# Autodesk Inventor assembly: Roof
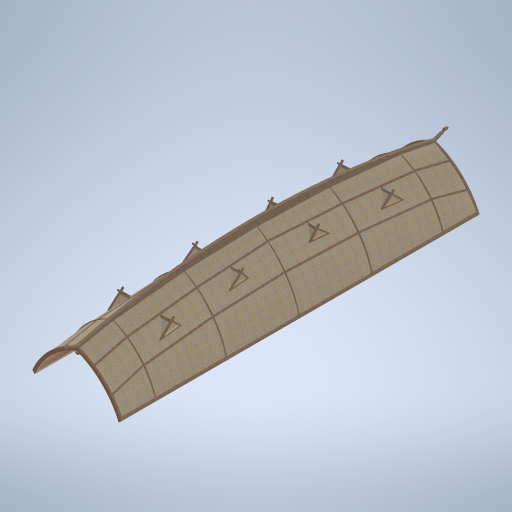
[picture p0: Inventor's stored thumbnail of the model, 512x512]
Saved by Autodesk Inventor 2024.2 (Build 282272000, 272)
## iProperties
Created: 2024-05-18
Part Number: Roof
Document SubType Name: Assembly
Designer: LOSTER_1
Author: LOSTER_1
## Documents named in this file (69)
- C:\Users\LOSTER_1\OneDrive\桌面\school\senior\Inventor_Project\ROOF\Roof.iam
- C:\Users\LOSTER_1\OneDrive\桌面\school\senior\Inventor_Project\ROOF\roof_beam.ipt
- C:\Users\LOSTER_1\OneDrive\桌面\school\senior\Inventor_Project\ROOF\gripping_beast.ipt
- C:\Users\LOSTER_1\OneDrive\桌面\school\senior\Inventor_Project\ROOF\main_crossbeam.ipt
- C:\Users\LOSTER_1\OneDrive\桌面\school\senior\Inventor_Project\ROOF\outer_curve_beam.ipt
- C:\Users\LOSTER_1\OneDrive\桌面\school\senior\Inventor_Project\ROOF\roof_straight_beam.ipt
- C:\Users\LOSTER_1\OneDrive\桌面\school\senior\Inventor_Project\ROOF\curve_beam_01.ipt
- C:\Users\LOSTER_1\OneDrive\桌面\school\senior\Inventor_Project\ROOF\curve_beam_02.ipt
- C:\Users\LOSTER_1\OneDrive\桌面\school\senior\Inventor_Project\ROOF\curve_beam_03.ipt
- C:\Users\LOSTER_1\OneDrive\桌面\school\senior\Inventor_Project\ROOF\support_beam_segments\support_beam_segment_0101.ipt
- C:\Users\LOSTER_1\OneDrive\桌面\school\senior\Inventor_Project\ROOF\support_beam_segments\support_beam_segment_0102.ipt
- C:\Users\LOSTER_1\OneDrive\桌面\school\senior\Inventor_Project\ROOF\support_beam_segments\support_beam_segment_0103.ipt
- C:\Users\LOSTER_1\OneDrive\桌面\school\senior\Inventor_Project\ROOF\support_beam_segments\support_beam_segment_0104.ipt
- C:\Users\LOSTER_1\OneDrive\桌面\school\senior\Inventor_Project\ROOF\support_beam_segments\support_beam_segment_0105.ipt
- C:\Users\LOSTER_1\OneDrive\桌面\school\senior\Inventor_Project\ROOF\support_beam_segments\support_beam_segment_0106.ipt
- C:\Users\LOSTER_1\OneDrive\桌面\school\senior\Inventor_Project\ROOF\support_beam_segments\support_beam_segment_0101_MIR.ipt
- C:\Users\LOSTER_1\OneDrive\桌面\school\senior\Inventor_Project\ROOF\support_beam_segments\support_beam_segment_0102_MIR.ipt
- C:\Users\LOSTER_1\OneDrive\桌面\school\senior\Inventor_Project\ROOF\support_beam_segments\support_beam_segment_0103_MIR.ipt
- C:\Users\LOSTER_1\OneDrive\桌面\school\senior\Inventor_Project\ROOF\support_beam_segments\support_beam_segment_0104_MIR.ipt
- C:\Users\LOSTER_1\OneDrive\桌面\school\senior\Inventor_Project\ROOF\support_beam_segments\support_beam_segment_0105_MIR.ipt
- C:\Users\LOSTER_1\OneDrive\桌面\school\senior\Inventor_Project\ROOF\support_beam_segments\support_beam_segment_0106_MIR.ipt
- C:\Users\LOSTER_1\OneDrive\桌面\school\senior\Inventor_Project\ROOF\support_beam_segments\support_beam_segment_0101_MIR1.ipt
- C:\Users\LOSTER_1\OneDrive\桌面\school\senior\Inventor_Project\ROOF\support_beam_segments\support_beam_segment_0102_MIR1.ipt
- C:\Users\LOSTER_1\OneDrive\桌面\school\senior\Inventor_Project\ROOF\support_beam_segments\support_beam_segment_0103_MIR1.ipt
- C:\Users\LOSTER_1\OneDrive\桌面\school\senior\Inventor_Project\ROOF\support_beam_segments\support_beam_segment_0104_MIR1.ipt
- C:\Users\LOSTER_1\OneDrive\桌面\school\senior\Inventor_Project\ROOF\support_beam_segments\support_beam_segment_0105_MIR1.ipt
- C:\Users\LOSTER_1\OneDrive\桌面\school\senior\Inventor_Project\ROOF\support_beam_segments\support_beam_segment_0106_MIR1.ipt
- C:\Users\LOSTER_1\OneDrive\桌面\school\senior\Inventor_Project\ROOF\support_beam_segments\support_beam_segment_0101_MIR_MIR.ipt
- C:\Users\LOSTER_1\OneDrive\桌面\school\senior\Inventor_Project\ROOF\support_beam_segments\support_beam_segment_0102_MIR_MIR.ipt
- C:\Users\LOSTER_1\OneDrive\桌面\school\senior\Inventor_Project\ROOF\support_beam_segments\support_beam_segment_0103_MIR_MIR.ipt
- C:\Users\LOSTER_1\OneDrive\桌面\school\senior\Inventor_Project\ROOF\support_beam_segments\support_beam_segment_0104_MIR_MIR.ipt
- C:\Users\LOSTER_1\OneDrive\桌面\school\senior\Inventor_Project\ROOF\support_beam_segments\support_beam_segment_0105_MIR_MIR.ipt
- C:\Users\LOSTER_1\OneDrive\桌面\school\senior\Inventor_Project\ROOF\support_beam_segments\support_beam_segment_0106_MIR_MIR.ipt
- C:\Users\LOSTER_1\OneDrive\桌面\school\senior\Inventor_Project\ROOF\panel_blocks\panel_block_03.ipt
- C:\Users\LOSTER_1\OneDrive\桌面\school\senior\Inventor_Project\ROOF\panel_blocks\panel_block_02.ipt
- C:\Users\LOSTER_1\OneDrive\桌面\school\senior\Inventor_Project\ROOF\panel_blocks\panel_block_01.ipt
- C:\Users\LOSTER_1\OneDrive\桌面\school\senior\Inventor_Project\ROOF\panel_blocks\panel_block_03_MIR.ipt
- C:\Users\LOSTER_1\OneDrive\桌面\school\senior\Inventor_Project\ROOF\panel_blocks\panel_block_02_MIR.ipt
- C:\Users\LOSTER_1\OneDrive\桌面\school\senior\Inventor_Project\ROOF\panel_blocks\panel_block_01_MIR.ipt
- C:\Users\LOSTER_1\OneDrive\桌面\school\senior\Inventor_Project\ROOF\panel_blocks\panel_block_03_MIR1.ipt
- C:\Users\LOSTER_1\OneDrive\桌面\school\senior\Inventor_Project\ROOF\panel_blocks\panel_block_01_MIR1.ipt
- C:\Users\LOSTER_1\OneDrive\桌面\school\senior\Inventor_Project\ROOF\panel_blocks\panel_block_03_MIR_MIR.ipt
- C:\Users\LOSTER_1\OneDrive\桌面\school\senior\Inventor_Project\ROOF\panel_blocks\panel_block_02_MIR_MIR.ipt
- C:\Users\LOSTER_1\OneDrive\桌面\school\senior\Inventor_Project\ROOF\panel_blocks\panel_block_01_MIR_MIR.ipt
- C:\Users\LOSTER_1\OneDrive\桌面\school\senior\Inventor_Project\ROOF\panel_blocks\panel_pad_02 .ipt
- C:\Users\LOSTER_1\OneDrive\桌面\school\senior\Inventor_Project\ROOF\panel_blocks\panel_block_02_MIR2.ipt
- C:\Users\LOSTER_1\OneDrive\桌面\school\senior\Inventor_Project\ROOF\panel_blocks\panel_pad_03.ipt
- C:\Users\LOSTER_1\OneDrive\桌面\school\senior\Inventor_Project\ROOF\panel_blocks\panel_pad_frame_01.ipt
- C:\Users\LOSTER_1\OneDrive\桌面\school\senior\Inventor_Project\ROOF\panel_blocks\panel_pad_frame_02.ipt
- C:\Users\LOSTER_1\OneDrive\桌面\school\senior\Inventor_Project\ROOF\panel_blocks\panel_pad_02 _MIR.ipt
- C:\Users\LOSTER_1\OneDrive\桌面\school\senior\Inventor_Project\ROOF\panel_blocks\panel_pad_03_MIR.ipt
- C:\Users\LOSTER_1\OneDrive\桌面\school\senior\Inventor_Project\ROOF\panel_blocks\panel_pad_frame_01_MIR.ipt
- C:\Users\LOSTER_1\OneDrive\桌面\school\senior\Inventor_Project\ROOF\panel_blocks\panel_pad_frame_02_MIR.ipt
- C:\Users\LOSTER_1\OneDrive\桌面\school\senior\Inventor_Project\ROOF\panel_blocks\panel_pad_02 _MIR1.ipt
- C:\Users\LOSTER_1\OneDrive\桌面\school\senior\Inventor_Project\ROOF\panel_blocks\panel_pad_03_MIR1.ipt
- C:\Users\LOSTER_1\OneDrive\桌面\school\senior\Inventor_Project\ROOF\panel_blocks\panel_pad_frame_01_MIR1.ipt
- C:\Users\LOSTER_1\OneDrive\桌面\school\senior\Inventor_Project\ROOF\panel_blocks\panel_pad_frame_02_MIR1.ipt
- C:\Users\LOSTER_1\OneDrive\桌面\school\senior\Inventor_Project\ROOF\panel_blocks\panel_pad_02 _MIR_MIR.ipt
- C:\Users\LOSTER_1\OneDrive\桌面\school\senior\Inventor_Project\ROOF\panel_blocks\panel_pad_03_MIR_MIR.ipt
- C:\Users\LOSTER_1\OneDrive\桌面\school\senior\Inventor_Project\ROOF\panel_blocks\panel_pad_frame_01_MIR_MIR.ipt
- C:\Users\LOSTER_1\OneDrive\桌面\school\senior\Inventor_Project\ROOF\panel_blocks\panel_pad_frame_02_MIR_MIR.ipt
- C:\Users\LOSTER_1\OneDrive\桌面\school\senior\Inventor_Project\ROOF\panel_blocks\pad_outframe_02.ipt
- C:\Users\LOSTER_1\OneDrive\桌面\school\senior\Inventor_Project\ROOF\panel_blocks\pad_outframe_03.ipt
- C:\Users\LOSTER_1\OneDrive\桌面\school\senior\Inventor_Project\ROOF\panel_blocks\pad_outframe_02_MIR.ipt
- C:\Users\LOSTER_1\OneDrive\桌面\school\senior\Inventor_Project\ROOF\panel_blocks\pad_outframe_03_MIR.ipt
- C:\Users\LOSTER_1\OneDrive\桌面\school\senior\Inventor_Project\ROOF\panel_blocks\pad_outframe_02_MIR1.ipt
- C:\Users\LOSTER_1\OneDrive\桌面\school\senior\Inventor_Project\ROOF\panel_blocks\pad_outframe_03_MIR1.ipt
- C:\Users\LOSTER_1\OneDrive\桌面\school\senior\Inventor_Project\ROOF\panel_blocks\pad_outframe_02_MIR_MIR.ipt
- C:\Users\LOSTER_1\OneDrive\桌面\school\senior\Inventor_Project\ROOF\panel_blocks\pad_outframe_03_MIR_MIR.ipt
## Components (80 placed, 68 different names)
1. roof_beam:1 — Mate:1, Mate:2, Mate:3, Mate:4, Mate:5, Mate:6, Mate:7, Mate:8, Mate:31, Mate:32, Mate:33, Mate:34, Mate:35, Mate:36, Mate:37, Mate:38, Mate:39, Mate:40, Mate:41, Mate:42, Mate:43, Mate:44, Mate:45, Mate:46, Mate:47, Mate:48, Mate:49, Mate:50, Mate:51, Mate:52, Mate:53, Mate:54, Mate:55, Flush:2
2. gripping_beast:1 — Mate:1, Mate:2, Mate:3, Mate:4
3. gripping_beast:2 — Mate:5
4. main_crossbeam:1 — Mate:6, Mate:7, Mate:8, Mate:11, Mate:14, Mate:19, Mate:20, Mate:21, Mate:22
5. outer_curve_beam:1 — Mate:9, Mate:10, Mate:11, Mate:12, Mate:13, Mate:26, Mate:28, Mate:56, Mate:57, Mate:58, Mate:59, Mate:60, Mate:74
6. outer_curve_beam:2 — Mate:9, Mate:10, Mate:12, Mate:13, Mate:14, Mate:29, Mate:30, Mate:75, Mate:76, Mate:77, Mate:78
7. outer_curve_beam:3 — Mate:23, Mate:24, Mate:25, Mate:27, Mate:79, Mate:80, Mate:81
8. outer_curve_beam:4 — Mate:19, Mate:20, Mate:21, Mate:22, Mate:23, Mate:24, Mate:25, Mate:82, Mate:83, Mate:84, Mate:85
9. roof_straight_beam:1 — Mate:26, Mate:27, Mate:28
10. roof_straight_beam:2 — Mate:29, Mate:30
11. curve_beam_01:1 — Mate:31, Mate:32, Mate:33
12. curve_beam_01:2 — Mate:34, Mate:35, Mate:61, Mate:63, Mate:64, Mate:65
13. curve_beam_01:3 — Mate:36, Mate:37
14. curve_beam_01:4 — Mate:38, Mate:39
15. curve_beam_02:1 — Mate:43, Mate:44
16. curve_beam_02:2 — Mate:40, Mate:41, Mate:42
17. curve_beam_02:3 — Mate:45, Mate:46, Mate:47, Mate:62, Mate:66, Mate:67, Mate:68, Mate:69, Mate:70
18. curve_beam_02:4 — Mate:48, Mate:49, Mate:50
19. curve_beam_03:1 — Mate:51, Mate:52, Flush:1
20. curve_beam_03:2 — Mate:53, Mate:54, Mate:55
21. support_beam_segment_0101:1 — Mate:56, Mate:57, Mate:58, Mate:73
22. support_beam_segment_0102:1 — Mate:59, Mate:60
23. support_beam_segment_0103:1 — Mate:61, Mate:62, Mate:71, Mate:72
24. support_beam_segment_0104:1 — Mate:63, Mate:64, Mate:65
25. support_beam_segment_0105:1 — Mate:66, Mate:67
26. support_beam_segment_0106:1 — Mate:68, Mate:69
27. support_beam_segment_0101_MIR:1 — Mate:80, Mate:81
28. support_beam_segment_0102_MIR:1 — Mate:79
29. support_beam_segment_0103_MIR:1
30. support_beam_segment_0104_MIR:1
31. support_beam_segment_0105_MIR:1
32. support_beam_segment_0106_MIR:1
33. support_beam_segment_0101_MIR1:1 — Mate:75, Mate:76
34. support_beam_segment_0102_MIR1:1 — Mate:77, Mate:78
35. support_beam_segment_0103_MIR1:1
36. support_beam_segment_0104_MIR1:1
37. support_beam_segment_0105_MIR1:1
38. support_beam_segment_0106_MIR1:1
39. support_beam_segment_0101_MIR_MIR:1 — Mate:82, Mate:83
40. support_beam_segment_0102_MIR_MIR:1 — Mate:84, Mate:85
41. support_beam_segment_0103_MIR_MIR:1
42. support_beam_segment_0104_MIR_MIR:1
43. support_beam_segment_0105_MIR_MIR:1
44. support_beam_segment_0106_MIR_MIR:1
45. panel_block_03:1 — Mate:70, Mate:87
46. panel_block_02:1 — Mate:71, Mate:72, Mate:86
47. panel_block_01:1 — Mate:73, Mate:74
48. panel_block_03_MIR:1
49. panel_block_02_MIR:1
50. panel_block_01_MIR:1
51. panel_block_03_MIR1:1
52. panel_block_01_MIR1:1
53. panel_block_03_MIR_MIR:1
54. panel_block_02_MIR_MIR:1
55. panel_block_01_MIR_MIR:1
56. panel_pad_02 :1 — Mate:86, Mate:88, Mate:96
57. panel_block_02_MIR2:1
58. panel_pad_03:1 — Mate:87, Mate:89
59. panel_pad_frame_01:1 — Mate:88
60. panel_pad_frame_02:1 — Mate:89, Mate:97
61. panel_pad_02 _MIR:1 — Mate:90
62. panel_pad_03_MIR:1 — Mate:91
63. panel_pad_frame_01_MIR:1 — Mate:90
64. panel_pad_frame_02_MIR:1 — Mate:91
65. panel_pad_02 _MIR1:1 — Mate:92
66. panel_pad_03_MIR1:1 — Mate:93
67. panel_pad_frame_01_MIR1:1 — Mate:92
68. panel_pad_frame_02_MIR1:1 — Mate:93
69. panel_pad_02 _MIR_MIR:1 — Mate:94
70. panel_pad_03_MIR_MIR:1 — Mate:95
71. panel_pad_frame_01_MIR_MIR:1 — Mate:94
72. panel_pad_frame_02_MIR_MIR:1 — Mate:95
73. pad_outframe_02:1 — Mate:96
74. pad_outframe_03:1 — Mate:97
75. pad_outframe_02_MIR:1
76. pad_outframe_03_MIR:1
77. pad_outframe_02_MIR1:1
78. pad_outframe_03_MIR1:1
79. pad_outframe_02_MIR_MIR:1
80. pad_outframe_03_MIR_MIR:1
## Relationships (99: Mate 97, Flush 2)
- Mate:1: roof_beam:1 ↔ gripping_beast:1
- Mate:2: roof_beam:1 ↔ gripping_beast:1
- Mate:3: roof_beam:1 ↔ gripping_beast:1
- Mate:4: roof_beam:1 ↔ gripping_beast:1
- Mate:5: roof_beam:1 ↔ gripping_beast:2
- Mate:6: roof_beam:1 ↔ main_crossbeam:1
- Mate:7: roof_beam:1 ↔ main_crossbeam:1
- Mate:8: roof_beam:1 ↔ main_crossbeam:1
- Mate:9: outer_curve_beam:1 ↔ outer_curve_beam:2
- Mate:10: outer_curve_beam:1 ↔ outer_curve_beam:2
- Mate:11: main_crossbeam:1 ↔ outer_curve_beam:1
- Mate:12: outer_curve_beam:1 ↔ outer_curve_beam:2
- Mate:13: outer_curve_beam:1 ↔ outer_curve_beam:2
- Mate:14: main_crossbeam:1 ↔ outer_curve_beam:2
- [Mate]: outer_curve_beam:3 ↔ outer_curve_beam:4
- [Mate]: outer_curve_beam:3 ↔ outer_curve_beam:4
- [Mate]: outer_curve_beam:3 ↔ outer_curve_beam:4
- [Mate]: outer_curve_beam:3 ↔ outer_curve_beam:4
- Mate:19: main_crossbeam:1 ↔ outer_curve_beam:4
- Mate:20: main_crossbeam:1 ↔ outer_curve_beam:4
- Mate:21: main_crossbeam:1 ↔ outer_curve_beam:4
- Mate:22: main_crossbeam:1 ↔ outer_curve_beam:4
- Mate:23: outer_curve_beam:3 ↔ outer_curve_beam:4
- Mate:24: outer_curve_beam:3 ↔ outer_curve_beam:4
- Mate:25: outer_curve_beam:3 ↔ outer_curve_beam:4
- Mate:26: outer_curve_beam:1 ↔ roof_straight_beam:1
- Mate:27: outer_curve_beam:3 ↔ roof_straight_beam:1
- Mate:28: outer_curve_beam:1 ↔ roof_straight_beam:1
- Mate:29: outer_curve_beam:2 ↔ roof_straight_beam:2
- Mate:30: outer_curve_beam:2 ↔ roof_straight_beam:2
- Mate:31: roof_beam:1 ↔ curve_beam_01:1
- Mate:32: roof_beam:1 ↔ curve_beam_01:1
- Mate:33: roof_beam:1 ↔ curve_beam_01:1
- Mate:34: roof_beam:1 ↔ curve_beam_01:2
- Mate:35: roof_beam:1 ↔ curve_beam_01:2
- Mate:36: roof_beam:1 ↔ curve_beam_01:3
- Mate:37: roof_beam:1 ↔ curve_beam_01:3
- Mate:38: roof_beam:1 ↔ curve_beam_01:4
- Mate:39: roof_beam:1 ↔ curve_beam_01:4
- Mate:40: roof_beam:1 ↔ curve_beam_02:2
- Mate:41: roof_beam:1 ↔ curve_beam_02:2
- Mate:42: roof_beam:1 ↔ curve_beam_02:2
- Mate:43: roof_beam:1 ↔ curve_beam_02:1
- Mate:44: roof_beam:1 ↔ curve_beam_02:1
- Mate:45: roof_beam:1 ↔ curve_beam_02:3
- Mate:46: roof_beam:1 ↔ curve_beam_02:3
- Mate:47: roof_beam:1 ↔ curve_beam_02:3
- Mate:48: roof_beam:1 ↔ curve_beam_02:4
- Mate:49: roof_beam:1 ↔ curve_beam_02:4
- Mate:50: roof_beam:1 ↔ curve_beam_02:4
- Mate:51: roof_beam:1 ↔ curve_beam_03:1
- Mate:52: roof_beam:1 ↔ curve_beam_03:1
- Mate:53: roof_beam:1 ↔ curve_beam_03:2
- Mate:54: roof_beam:1 ↔ curve_beam_03:2
- Mate:55: roof_beam:1 ↔ curve_beam_03:2
- Mate:56: outer_curve_beam:1 ↔ support_beam_segment_0101:1
- Mate:57: outer_curve_beam:1 ↔ support_beam_segment_0101:1
- Mate:58: outer_curve_beam:1 ↔ support_beam_segment_0101:1
- Mate:59: outer_curve_beam:1 ↔ support_beam_segment_0102:1
- Mate:60: outer_curve_beam:1 ↔ support_beam_segment_0102:1
- Mate:61: curve_beam_01:2 ↔ support_beam_segment_0103:1
- Mate:62: curve_beam_02:3 ↔ support_beam_segment_0103:1
- Mate:63: curve_beam_01:2 ↔ support_beam_segment_0104:1
- Mate:64: curve_beam_01:2 ↔ support_beam_segment_0104:1
- Mate:65: curve_beam_01:2 ↔ support_beam_segment_0104:1
- Mate:66: curve_beam_02:3 ↔ support_beam_segment_0105:1
- Mate:67: curve_beam_02:3 ↔ support_beam_segment_0105:1
- Mate:68: curve_beam_02:3 ↔ support_beam_segment_0106:1
- Mate:69: curve_beam_02:3 ↔ support_beam_segment_0106:1
- Flush:1 (-50 mm): curve_beam_03:1
- Flush:2 (-150 mm): roof_beam:1
- Mate:70: curve_beam_02:3 ↔ panel_block_03:1
- Mate:71: support_beam_segment_0103:1 ↔ panel_block_02:1
- Mate:72: support_beam_segment_0103:1 ↔ panel_block_02:1
- Mate:73: support_beam_segment_0101:1 ↔ panel_block_01:1
- Mate:74: outer_curve_beam:1 ↔ panel_block_01:1
- Mate:75: outer_curve_beam:2 ↔ support_beam_segment_0101_MIR1:1
- Mate:76: outer_curve_beam:2 ↔ support_beam_segment_0101_MIR1:1
- Mate:77: outer_curve_beam:2 ↔ support_beam_segment_0102_MIR1:1
- Mate:78: outer_curve_beam:2 ↔ support_beam_segment_0102_MIR1:1
- Mate:79: outer_curve_beam:3 ↔ support_beam_segment_0102_MIR:1
- Mate:80: outer_curve_beam:3 ↔ support_beam_segment_0101_MIR:1
- Mate:81: outer_curve_beam:3 ↔ support_beam_segment_0101_MIR:1
- Mate:82: outer_curve_beam:4 ↔ support_beam_segment_0101_MIR_MIR:1
- Mate:83: outer_curve_beam:4 ↔ support_beam_segment_0101_MIR_MIR:1
- Mate:84: outer_curve_beam:4 ↔ support_beam_segment_0102_MIR_MIR:1
- Mate:85: outer_curve_beam:4 ↔ support_beam_segment_0102_MIR_MIR:1
- Mate:86: panel_block_02:1 ↔ panel_pad_02 :1
- Mate:87: panel_block_03:1 ↔ panel_pad_03:1
- Mate:88: panel_pad_02 :1 ↔ panel_pad_frame_01:1
- Mate:89: panel_pad_03:1 ↔ panel_pad_frame_02:1
- Mate:90: panel_pad_02 _MIR:1 ↔ panel_pad_frame_01_MIR:1
- Mate:91: panel_pad_03_MIR:1 ↔ panel_pad_frame_02_MIR:1
- Mate:92: panel_pad_02 _MIR1:1 ↔ panel_pad_frame_01_MIR1:1
- Mate:93: panel_pad_03_MIR1:1 ↔ panel_pad_frame_02_MIR1:1
- Mate:94: panel_pad_02 _MIR_MIR:1 ↔ panel_pad_frame_01_MIR_MIR:1
- Mate:95: panel_pad_03_MIR_MIR:1 ↔ panel_pad_frame_02_MIR_MIR:1
- Mate:96: panel_pad_02 :1 ↔ pad_outframe_02:1
- Mate:97: panel_pad_frame_02:1 ↔ pad_outframe_03:1
## Named parameters: d16_d10 = 0 mm, d17_d11 = 0 mm, d18_d13 = 0 mm, d19_d14 = 0 mm
